# Autodesk Inventor assembly: A_ankle_wing_001
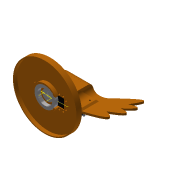
[picture p0: Inventor's stored thumbnail of the model, 180x180]
Saved by Autodesk Inventor 2016 (Build 200138000, 138)
## iProperties
Created: 2016-02-23
Part Number: A_ankle_wing_001
Document SubType Name: Assembly
Designer: Mateusz
Author: Mateusz
## Documents named in this file (9)
- D:\PROJECTS\2016_biped\hermes\mechanics_tmp\A_ankle_wing_001.iam
- D:\PROJECTS\2016_biped\hermes\mechanics_tmp\AX-12A.iam
- D:\PROJECTS\2016_biped\hermes\mechanics_tmp\P_ankle01_001.ipt
- D:\PROJECTS\2016_biped\hermes\mechanics_tmp\P_bearing_Z9089_001.ipt
- D:\PROJECTS\2016_biped\hermes\mechanics_tmp\P_ankle02_001.ipt
- D:\PROJECTS\2016_biped\hermes\mechanics_tmp\SharpIRsensor.ipt
- D:\PROJECTS\2016_biped\hermes\mechanics_tmp\P_ankle02front_001.ipt
- D:\PROJECTS\2016_biped\hermes\mechanics_tmp\P_akle02back_001.ipt
- D:\PROJECTS\2016_biped\hermes\mechanics_tmp\P_ankle03_001.ipt
## Components (8 placed, 8 different names)
1. AX-12A:1 [sub-assembly] — Mate:1, Angle:1, Mate:2, Mate:3, Angle:2, Mate:5, Mate:21
2. P_ankle01_001:1 — Flush:1, Mate:3, Mate:5, Mate:6, Mate:8, Tangent:1, Mate:21
3. P_bearing_Z9089_001:1 — Mate:6, Mate:7
4. P_ankle02_001:1 — Mate:11, Mate:12, Mate:13
5. SharpIRsensor:1 — Mate:18, Tangent:1, Mate:19
6. P_ankle02front_001:1 — Mate:8, Mate:10, Mate:17
7. P_ankle02back_001:1 — Mate:14, Mate:15, Mate:16, Mate:18, Mate:19, Mate:20, Insert:1
8. P_ankle03_001:1 — Mate:20, Insert:1
## Relationships (24: Mate 19, Angle 2, Flush 1, Tangent 1, Insert 1)
- Mate:1: AX-12A:1
- Angle:1 (0 deg): AX-12A:1
- Mate:2: AX-12A:1
- Flush:1: P_ankle01_001:1
- Mate:3: AX-12A:1 ↔ P_ankle01_001:1
- Angle:2 (0 deg): AX-12A:1
- Mate:5: AX-12A:1 ↔ P_ankle01_001:1
- Mate:6: P_ankle01_001:1 ↔ P_bearing_Z9089_001:1
- Mate:7: P_bearing_Z9089_001:1
- Mate:8: P_ankle01_001:1 ↔ P_ankle02front_001:1
- Mate:10: P_ankle02front_001:1
- Mate:11: P_ankle02_001:1
- Mate:12: P_ankle02_001:1
- Mate:13: P_ankle02_001:1
- Mate:14: P_ankle02back_001:1
- Mate:15: P_ankle02back_001:1
- Mate:16: P_ankle02back_001:1
- Mate:17: P_ankle02front_001:1
- Mate:18: SharpIRsensor:1 ↔ P_ankle02back_001:1
- Tangent:1: P_ankle01_001:1 ↔ SharpIRsensor:1
- Mate:19: SharpIRsensor:1 ↔ P_ankle02back_001:1
- Mate:20: P_ankle02back_001:1 ↔ P_ankle03_001:1
- Insert:1: P_ankle02back_001:1 ↔ P_ankle03_001:1
- Mate:21: AX-12A:1 ↔ P_ankle01_001:1
